# Autodesk Inventor assembly: Сборка1
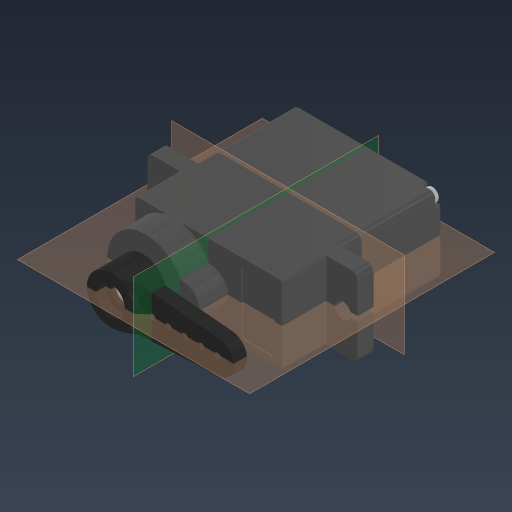
[picture p0: Inventor's stored thumbnail of the model, 512x512]
Saved by Autodesk Inventor 2023.2 (Build 272271030, 271C)
## iProperties
Created: 2026-01-05
Part Number: Сборка1
Document SubType Name: Assembly
Designer: Олег Коноваленко
Author: Олег Коноваленко
## Documents named in this file (3)
- D:\VSOSH_IT_Robotics_ETZ\ETZ\Сonstruction\Сборка1.iam
- D:\VSOSH_IT_Robotics_ETZ\ETZ\Сonstruction\Качалка.ipt
- D:\VSOSH_IT_Robotics_ETZ\ETZ\Сonstruction\MG90S Micro Servo Motor.ipt
## Components (2 placed, 2 different names)
1. Качалка:1 — Совмещение:1, Совмещение:2
2. MG90S Micro Servo Motor:1 — Совмещение:1, Совмещение:2, Совмещение:3, Заподлицо:1, Заподлицо:2
## Relationships (5: Mate 3, Flush 2)
- Совмещение:1 [Mate]: Качалка:1 ↔ MG90S Micro Servo Motor:1
- Совмещение:2 [Mate]: Качалка:1 ↔ MG90S Micro Servo Motor:1
- Совмещение:3 [Mate]: MG90S Micro Servo Motor:1
- Заподлицо:1 [Flush]: MG90S Micro Servo Motor:1
- Заподлицо:2 [Flush]: MG90S Micro Servo Motor:1
